# Autodesk Inventor assembly: buggy-assembly-group2
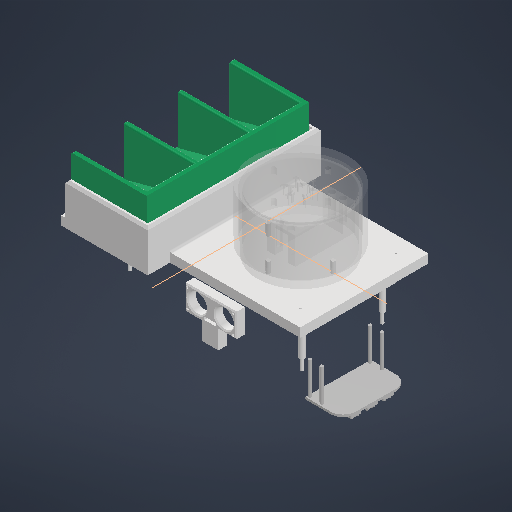
[picture p0: Inventor's stored thumbnail of the model, 512x512]
Saved by Autodesk Inventor 2026.1 (Build 301233000, 233)
## iProperties
Created: 2026-02-23
Part Number: buggy-assembly-group2
Document SubType Name: Assembly
Designer: ts2104
Author: ts2104
## Documents named in this file (6)
- C:\Git\System-Project-G2\mechanical\buggy-assembly-group2.iam
- C:\Git\System-Project-G2\mechanical\rubbish-container-group2.ipt
- C:\Git\System-Project-G2\mechanical\crane-base-assembly.iam
- C:\Git\System-Project-G2\mechanical\buggy-body-assembly-ready-group2.ipt
- C:\Git\System-Project-G2\mechanical\line-follower-group2.ipt
- C:\Git\System-Project-G2\mechanical\us-sensor-mount.ipt
## Components (5 placed, 5 different names)
1. rubbish-container-group2:1 — Flush:1, Mate:4
2. crane-base-assembly:1 [sub-assembly] — Mate:5, Mate:6
3. buggy-body-assembly-ready-group2:1 — Mate:1, Mate:2, Mate:3, Mate:4, Mate:5, Mate:8, Mate:9
4. line-follower-group2:1
5. us-sensor-mount:1 — Mate:8, Mate:9
## Relationships (9: Mate 8, Flush 1)
- Mate:1: buggy-body-assembly-ready-group2:1
- Mate:2: buggy-body-assembly-ready-group2:1
- Mate:3: buggy-body-assembly-ready-group2:1
- Flush:1: rubbish-container-group2:1
- Mate:4: rubbish-container-group2:1 ↔ buggy-body-assembly-ready-group2:1
- Mate:5: crane-base-assembly:1 ↔ buggy-body-assembly-ready-group2:1
- Mate:6: crane-base-assembly:1
- Mate:8: buggy-body-assembly-ready-group2:1 ↔ us-sensor-mount:1
- Mate:9: buggy-body-assembly-ready-group2:1 ↔ us-sensor-mount:1
